# Autodesk Inventor assembly: platforma
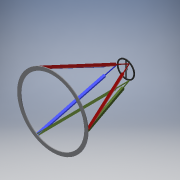
[picture p0: Inventor's stored thumbnail of the model, 180x180]
Saved by Autodesk Inventor 2017 (Build 210142000, 142)
## iProperties
Created: 2016-07-21
Part Number: platforma
Document SubType Name: Assembly
Designer: Marcin
Mass: 907726 g
Surface Area: 61088.9 cm^2
Volume: 119965 cm^3
Density: 7.56657 g/cm^3
Author: Marcin
## Documents named in this file (6)
- M:\PracaInżynierska\platforma.iam
- M:\PracaInżynierska\Part1.ipt
- M:\PracaInżynierska\platforma.ipt
- M:\PracaInżynierska\Aktutator.iam
- M:\PracaInżynierska\KinematicMidWay.ipt
- M:\PracaInżynierska\sitting_dummy_1_76_m_22111111611.ipt
## Components (10 placed, 5 different names)
1. Part1:1 — akt_podstawa_01, akt_podstawa_02, akt_podstawa_03, akt_podstawa_04, akt_podstawa_05, akt_podstawa_06
2. platforma:1 — Flush:1
3. Aktutator:1 [sub-assembly] — akt_podstawa_01
4. Aktutator:2 [sub-assembly] — akt_podstawa_02
5. Aktutator:3 [sub-assembly] — akt_podstawa_03
6. Aktutator:4 [sub-assembly] — akt_podstawa_04
7. Aktutator:5 [sub-assembly] — akt_podstawa_05
8. Aktutator:6 [sub-assembly] — akt_podstawa_06
9. KinematicMidWay:1 — Flush:1
10. sitting_dummy_1_76_m_22111111611:1
## Relationships (7: BallJoint 6, Flush 1)
- akt_podstawa_01 [BallJoint]: Part1:1 ↔ Aktutator:1
- akt_podstawa_02 [BallJoint]: Part1:1 ↔ Aktutator:2
- akt_podstawa_03 [BallJoint]: Part1:1 ↔ Aktutator:3
- akt_podstawa_04 [BallJoint]: Part1:1 ↔ Aktutator:4
- akt_podstawa_05 [BallJoint]: Part1:1 ↔ Aktutator:5
- akt_podstawa_06 [BallJoint]: Part1:1 ↔ Aktutator:6
- Flush:1: platforma:1 ↔ KinematicMidWay:1
